# Autodesk Inventor assembly: 117_MIR
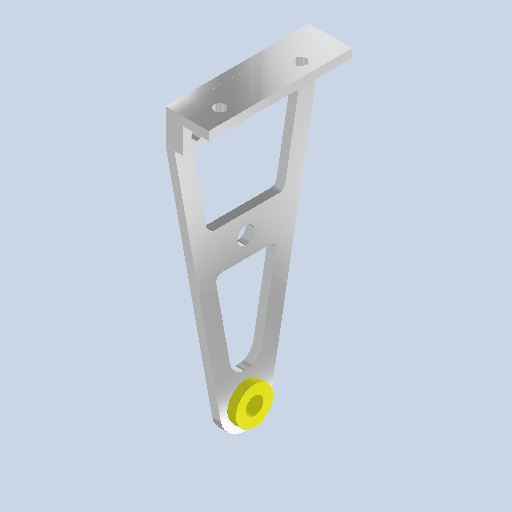
[picture p0: Inventor's stored thumbnail of the model, 512x512]
Saved by Autodesk Inventor 2025.1 (Build 291241000, 241)
## iProperties
Created: 2024-06-11
Part Number: 117_MIR
Document SubType Name: Assembly
Designer: ffogue
Author: ffogue
## Documents named in this file (4)
- C:\Users\ffogue\Downloads\Meine Projket\Paddle\117_MIR.iam
- C:\Users\ffogue\Downloads\Meine Projket\Paddle\1171_MIR.ipt
- C:\Users\ffogue\Downloads\Meine Projket\Paddle\1172_MIR.ipt
- C:\Users\ffogue\Downloads\Meine Projket\Paddle\1173_MIR.ipt
## Components (3 placed, 1 different names)
1. Supporttriangle:1 — Insert:1, Insert:2
2. Supporttriangle:2 — Insert:1
3. Supporttriangle:3 — Insert:2
## Relationships (2: Insert 2)
- Insert:1: Supporttriangle:1 ↔ Supporttriangle:2
- Insert:2: Supporttriangle:1 ↔ Supporttriangle:3
